# Autodesk Inventor assembly: Feeder Assembly
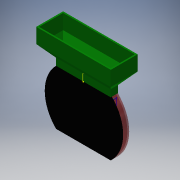
[picture p0: Inventor's stored thumbnail of the model, 180x180]
Saved by Autodesk Inventor 2017 (Build 210142000, 142)
## iProperties
Created: 2018-12-13
Part Number: Feeder Assembly
Document SubType Name: Assembly
Designer: Matt
Author: Matt
## Documents named in this file (6)
- C:\Users\Matt\Documents\Cat Feeder\Feeder Assembly.iam
- C:\Users\Matt\Documents\Cat Feeder\nema 17 stepper motor (triple stack).ipt
- C:\Users\Matt\Documents\Cat Feeder\Dispensing Gear.ipt
- C:\Users\Matt\Documents\Cat Feeder\Gear Container.ipt
- C:\Users\Matt\Documents\Cat Feeder\Gear Container Lid.ipt
- C:\Users\Matt\Documents\Cat Feeder\Food Holder.ipt
## Components (5 placed, 5 different names)
1. nema 17 stepper motor (triple stack):1 — Insert:1, Insert:2
2. Dispensing Gear:1 — Insert:2
3. Gear Container:1 — Insert:1, Mate:2, Mate:3, Mate:4
4. Gear Container Lid:1 — Mate:2, Mate:3, Mate:5
5. Food Holder:1 — Mate:4, Mate:5
## Relationships (6: Mate 4, Insert 2)
- Insert:1 (16.51 mm): nema 17 stepper motor (triple stack):1 ↔ Gear Container:1
- Mate:2: Gear Container:1 ↔ Gear Container Lid:1
- Insert:2 (-13.97 mm): nema 17 stepper motor (triple stack):1 ↔ Dispensing Gear:1
- Mate:3: Gear Container:1 ↔ Gear Container Lid:1
- Mate:4: Gear Container:1 ↔ Food Holder:1
- Mate:5: Gear Container Lid:1 ↔ Food Holder:1
